# Autodesk Inventor assembly: bevel gear with clamping hub_MIR
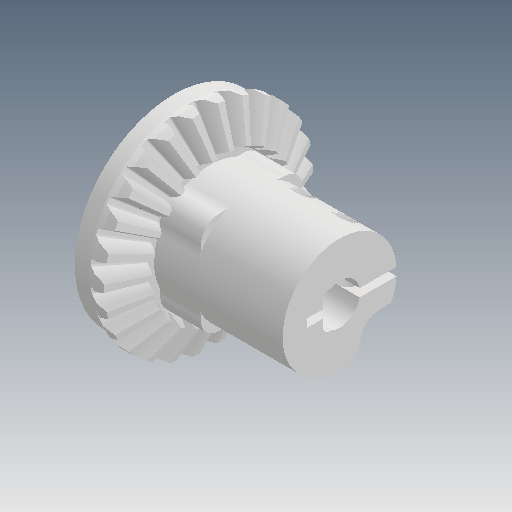
[picture p0: Inventor's stored thumbnail of the model, 512x512]
Saved by Autodesk Inventor 2020 (Build 240168000, 168)
## iProperties
Created: 2019-09-29
Part Number: bevel gear with clamping hub_MIR
Document SubType Name: Assembly
Designer: ball
Author: ball
## Documents named in this file (4)
- C:\FTC\FTC8863CAD\2019 Robot\Mecanum Drive Train\bevel gear with clamping hub_MIR.iam
- C:\FTC\FTC8863CAD\Actobotics\615 parts\615460_MIR.ipt
- C:\FTC\FTC8863CAD\Actobotics\545 parts\545309_MIR.ipt
- C:\FTC\FTC8863CAD\Actobotics\632 parts\632108_MIR.ipt
## Components (6 placed, 3 different names)
1. 615460_MIR:1 — Mate:3, Mate:2, Mate:1, Mate:5, Mate:4, Mate:7, Mate:8, Mate:6
2. 545309_MIR:1 — Mate:3, Mate:2, Mate:1, Mate:11, Mate:10, Mate:9
3. 632108_MIR:1 — Mate:5, Mate:4
4. 632108_MIR:2 — Mate:11, Mate:7
5. 632108_MIR:3 — Mate:10, Mate:8
6. 632108_MIR:4 — Mate:9, Mate:6
## Relationships (11: Mate 11)
- Mate:3: 615460_MIR:1 ↔ 545309_MIR:1
- Mate:2: 615460_MIR:1 ↔ 545309_MIR:1
- Mate:1: 615460_MIR:1 ↔ 545309_MIR:1
- Mate:5: 615460_MIR:1 ↔ 632108_MIR:1
- Mate:4: 615460_MIR:1 ↔ 632108_MIR:1
- Mate:11: 545309_MIR:1 ↔ 632108_MIR:2
- Mate:7: 615460_MIR:1 ↔ 632108_MIR:2
- Mate:10: 545309_MIR:1 ↔ 632108_MIR:3
- Mate:8: 615460_MIR:1 ↔ 632108_MIR:3
- Mate:9: 545309_MIR:1 ↔ 632108_MIR:4
- Mate:6: 615460_MIR:1 ↔ 632108_MIR:4
